# Autodesk Inventor assembly: Assy_linear_module
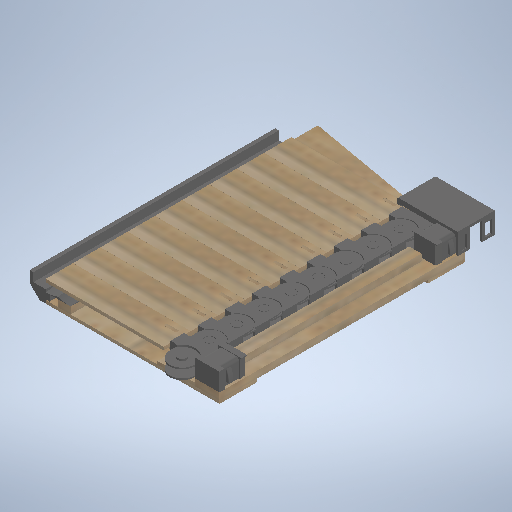
[picture p0: Inventor's stored thumbnail of the model, 512x512]
Saved by Autodesk Inventor 2026.1 (Build 301233020, 233B)
## iProperties
Created: 2025-09-27
Part Number: Assy_linear_module
Document SubType Name: Assembly
Designer: hibik
Author: hibik
## Documents named in this file (10)
- C:\Users\hibik\Documents\Robomech\conveyer\liniar_module\Assy_linear_module.iam
- C:\Users\hibik\Documents\Robomech\conveyer\liniar_module\base.ipt
- C:\Users\hibik\Documents\Robomech\conveyer\liniar_module\connector_base.ipt
- C:\Users\hibik\Documents\Robomech\conveyer\liniar_module\back_upper.ipt
- C:\Users\hibik\Documents\Robomech\conveyer\connector_module\connector_male.ipt
- C:\Users\hibik\Documents\Robomech\conveyer\liniar_module\belt_rail.ipt
- C:\Users\hibik\Documents\Robomech\conveyer\liniar_module\front.ipt
- C:\Users\hibik\Documents\Robomech\conveyer\belt\belt_linear.iam
- C:\Users\hibik\Documents\Robomech\conveyer\liniar_module\front_rail.ipt
- C:\Users\hibik\Documents\Robomech\conveyer\connectors\connetcor_female_cover.ipt
## Components (11 placed, 9 different names)
1. base:1 — メイト:1, フラッシュ:1, フラッシュ:3, メイト:7, フラッシュ:7, フラッシュ:8, フラッシュ:9, メイト:12, フラッシュ:11
2. connector_base:1 — メイト:1, フラッシュ:1, フラッシュ:3, メイト:3, フラッシュ:5, フラッシュ:6, メイト:4, メイト:5, メイト:6, メイト:8, メイト:9, メイト:10, メイト:11, メイト:13, メイト:14
3. base:2 — メイト:3, フラッシュ:5, フラッシュ:6
4. connector_male:7 — メイト:9, メイト:10, メイト:11, メイト:16
5. connector_male:8 — メイト:4, メイト:5, メイト:6
6. belt_rail:1 — メイト:7, フラッシュ:7, メイト:8, 正接:1, 角度:1
7. front:1 — フラッシュ:8, フラッシュ:9, メイト:12, フラッシュ:12, フラッシュ:13, フラッシュ:14
8. back_upper:1 — フラッシュ:10, メイト:13, メイト:14, メイト:15
9. belt_linear:1 [sub-assembly] — メイト:15, 正接:1, 角度:1, フラッシュ:11
10. front_rail:1 — フラッシュ:12, フラッシュ:13, フラッシュ:14
11. connetcor_female_cover:1 — メイト:16
## Relationships (29: Mate 15, Flush 12, Tangent 1, Angle 1)
- メイト:1 [Mate]: base:1 ↔ connector_base:1
- フラッシュ:1 [Flush]: base:1 ↔ connector_base:1
- フラッシュ:3 [Flush]: base:1 ↔ connector_base:1
- メイト:3 [Mate]: connector_base:1 ↔ base:2
- フラッシュ:5 [Flush]: connector_base:1 ↔ base:2
- フラッシュ:6 [Flush]: connector_base:1 ↔ base:2
- メイト:4 [Mate]: connector_base:1 ↔ connector_male:8
- メイト:5 [Mate]: connector_base:1 ↔ connector_male:8
- メイト:6 [Mate]: connector_base:1 ↔ connector_male:8
- メイト:7 [Mate]: base:1 ↔ belt_rail:1
- フラッシュ:7 [Flush]: base:1 ↔ belt_rail:1
- メイト:8 [Mate]: connector_base:1 ↔ belt_rail:1
- メイト:9 [Mate]: connector_base:1 ↔ connector_male:7
- メイト:10 [Mate]: connector_base:1 ↔ connector_male:7
- メイト:11 [Mate]: connector_base:1 ↔ connector_male:7
- フラッシュ:8 [Flush]: base:1 ↔ front:1
- フラッシュ:9 [Flush]: base:1 ↔ front:1
- メイト:12 [Mate]: base:1 ↔ front:1
- フラッシュ:10 [Flush]: back_upper:1
- メイト:13 [Mate]: connector_base:1 ↔ back_upper:1
- メイト:14 [Mate]: connector_base:1 ↔ back_upper:1
- メイト:15 [Mate]: back_upper:1 ↔ belt_linear:1
- 正接:1 [Tangent]: belt_rail:1 ↔ belt_linear:1
- 角度:1 [Angle] (0 deg): belt_rail:1 ↔ belt_linear:1
- フラッシュ:11 [Flush]: base:1 ↔ belt_linear:1
- フラッシュ:12 [Flush]: front:1 ↔ front_rail:1
- フラッシュ:13 [Flush]: front:1 ↔ front_rail:1
- フラッシュ:14 [Flush]: front:1 ↔ front_rail:1
- メイト:16 [Mate]: connector_male:7 ↔ connetcor_female_cover:1
